# Autodesk Inventor assembly: RoomboticsField2018
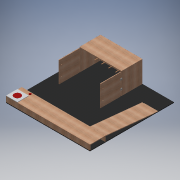
[picture p0: Inventor's stored thumbnail of the model, 180x180]
Saved by Autodesk Inventor 2019 (Build 230136000, 136)
## iProperties
Created: 2018-09-21
Part Number: RoomboticsField2018
Document SubType Name: Assembly
Designer: user
Author: user
## Documents named in this file (4)
- C:\Users\user\Desktop\Roombotics\RoomboticsField2018.iam
- C:\Users\user\Desktop\College\IPRO\SwerveProto\Base.ipt
- C:\Users\user\Desktop\Roombotics\Cabinet.iam
- C:\Users\user\Desktop\Roombotics\UpperLevel.iam
## Components (3 placed, 3 different names)
1. Base:1 — Flush:1, Mate:1, Flush:2, Flush:3, Flush:4, Mate:2
2. Cabinet:1 [sub-assembly] — Flush:1, Mate:1, Flush:2
3. UpperLevel:1 [sub-assembly] — Flush:3, Flush:4, Mate:2
## Relationships (6: Flush 4, Mate 2)
- Flush:1 (304.8 mm): Base:1 ↔ Cabinet:1
- Mate:1: Base:1 ↔ Cabinet:1
- Flush:2: Base:1 ↔ Cabinet:1
- Flush:3: Base:1 ↔ UpperLevel:1
- Flush:4: Base:1 ↔ UpperLevel:1
- Mate:2: Base:1 ↔ UpperLevel:1
